# Autodesk Inventor assembly: Horizontaly opening Door
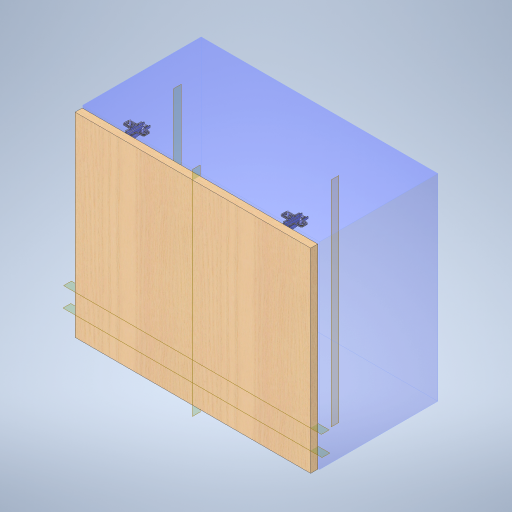
[picture p0: Inventor's stored thumbnail of the model, 512x512]
Saved by Autodesk Inventor 2024 (Build 280153000, 153)
## iProperties
RuleStatus: InUse
Created: 2017-01-20
Part Number: Horizontaly opening Door
Document SubType Name: Assembly
Designer: SvetlanaB
Description: Horizontaly opening Door
Author: SvetlanaB
## Documents named in this file (5)
- C:\W4INV 2024 Design\iBOX LIBRARY\Kitchen\Doors\Horizontaly opening Door\Horizontaly opening Door.iam
- C:\W4INV 2024 Design\iBOX LIBRARY\Kitchen\Doors\Horizontaly opening Door\Horizontaly opening Door.ipt
- C:\W4INV 2024 Design\iBOX LIBRARY\Kitchen\Doors\Horizontaly opening Door\Horizontaly opening Door skeleton.ipt
- C:\W4INV 2024 Design\_LIBRARY\Hinges\CONCEALED HINGE\Full Overlay Hinge Wood Screw Cup Wood Screw T18.iam
- C:\W4INV 2023 Design\LIBRARY\Hinges\CONCEALED HINGE.iam
## Components (4 placed, 3 different names)
1. @Skeleton — Flush:11, Flush:12, Flush:13, Flush:6, Flush:7, Flush:15, Flush:16
2. Horizontaly opening Door:1 — Flush:1, Mate:6, Angle:2, Mate:7, Mate:9, Flush:17
3. Full Overlay Hinge Wood Screw Cup Wood Screw T18:1 [sub-assembly] — Flush:14, Flush:15, Mate:7
4. Full Overlay Hinge Wood Screw Cup Wood Screw T18:2 [sub-assembly] — Mate:8, Flush:16, Mate:9
## Relationships (15: Flush 10, Mate 4, Angle 1)
- Flush:1 (-100 mm): Horizontaly opening Door:1
- Mate:6: Horizontaly opening Door:1
- Angle:2 (0 deg): Horizontaly opening Door:1
- Flush:6 (-100 mm): @Skeleton
- Flush:7 (-100 mm): @Skeleton
- Flush:11: @Skeleton
- Flush:12: @Skeleton
- Flush:13: @Skeleton
- Flush:14: Full Overlay Hinge Wood Screw Cup Wood Screw T18:1
- Flush:15 (18 mm): @Skeleton ↔ Full Overlay Hinge Wood Screw Cup Wood Screw T18:1
- Mate:7: Horizontaly opening Door:1 ↔ Full Overlay Hinge Wood Screw Cup Wood Screw T18:1
- Mate:8: Full Overlay Hinge Wood Screw Cup Wood Screw T18:2
- Flush:16 (18 mm): @Skeleton ↔ Full Overlay Hinge Wood Screw Cup Wood Screw T18:2
- Mate:9: Horizontaly opening Door:1 ↔ Full Overlay Hinge Wood Screw Cup Wood Screw T18:2
- Flush:17 (-50 mm): Horizontaly opening Door:1
## Named parameters: Heigth = 500 mm, Width = 600 mm, Side_allowance = 3 mm, Panel_thickness = 18 mm, Offset_L = 1.5 mm, Offset_R = 1.5 mm, Offset_Top = 4 mm, Offset_Bottom = 1.5 mm, Cupboard_Panel_Thickness = 18 mm
